# Autodesk Inventor assembly: RC_Car
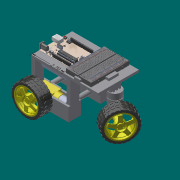
[picture p0: Inventor's stored thumbnail of the model, 180x180]
Saved by Autodesk Inventor 2019 (Build 230136000, 136)
## iProperties
Created: 2020-12-04
Part Number: RC_Car
Document SubType Name: Assembly
Designer: Jason
Mass: 430.82 g
Surface Area: 2607.9 cm^2
Volume: 430.82 cm^3
Density: 1 g/cm^3
Author: Jason
## Documents named in this file (11)
- D:\Inventor Files\RC_Car\RC_Car.iam
- D:\Inventor Files\RC_Car\Arduino Uno.ipt
- D:\Inventor Files\RC_Car\dc_motorl.ipt
- D:\Inventor Files\RC_Car\dc_wheel.ipt
- D:\Inventor Files\RC_Car\RC_Chassis.ipt
- D:\Inventor Files\RC_Car\breadboard_350_pos_asm.ipt
- D:\Inventor Files\RC_Car\BATTERY PACK BASE.ipt
- D:\Inventor Files\RC_Car\BATTERY PACK COVER.ipt
- D:\Inventor Files\RC_Car\Swing_Joint.ipt
- D:\Inventor Files\RC_Car\Swing_Joint_2.ipt
- D:\Inventor Files\RC_Car\Joint_Wheel_Connect.ipt
## Components (13 placed, 10 different names)
1. dc_motorl:1 — Mate:19, Flush:18, Mate:20, Insert:2
2. dc_motorl:2 — Flush:17, Mate:18, Mate:21, Insert:3
3. dc_wheel:2 — Insert:3
4. dc_wheel:3 — Insert:2
5. dc_wheel:1 — Mate:14, Mate:15, Mate:16
6. Arduino Uno:1 — Angle:6, Angle:7, Mate:24
7. BATTERY PACK COVER:1 — Mate:3, Mate:5, Mate:6, Mate:17, Flush:16
8. BATTERY PACK BASE:1 — Mate:3, Mate:5, Mate:6, Angle:6, Angle:7, Mate:23
9. breadboard_350_pos_asm:1 — Mate:9, Mate:10, Mate:22
10. RC_Chassis:1 — Mate:9, Mate:10, Flush:8, Flush:10, Mate:12, Flush:11, Mate:13, Mate:17, Flush:16, Flush:17, Mate:18, Mate:19, Flush:18, Mate:20, Mate:21, Mate:22, Mate:23, Mate:24
11. Swing_Joint:1 — Flush:8, Flush:10, Mate:12, Flush:11, Mate:13, Flush:12, Flush:13, Rotational:1
12. Swing_Joint_2:1 — Flush:12, Flush:13, Rotational:1, Flush:14, Flush:15
13. Joint_Wheel_Connect:1 — Flush:14, Flush:15, Mate:14, Mate:15, Mate:16
## Relationships (33: Mate 18, Flush 10, Angle 2, Insert 2, RevoluteJoint 1)
- Mate:3: BATTERY PACK COVER:1 ↔ BATTERY PACK BASE:1
- Mate:5: BATTERY PACK COVER:1 ↔ BATTERY PACK BASE:1
- Mate:6: BATTERY PACK COVER:1 ↔ BATTERY PACK BASE:1
- Angle:6 (0 deg): Arduino Uno:1 ↔ BATTERY PACK BASE:1
- Angle:7 (0 deg): Arduino Uno:1 ↔ BATTERY PACK BASE:1
- Mate:9: breadboard_350_pos_asm:1 ↔ RC_Chassis:1
- Mate:10: breadboard_350_pos_asm:1 ↔ RC_Chassis:1
- Flush:8: RC_Chassis:1 ↔ Swing_Joint:1
- Flush:10 (12.7 mm): RC_Chassis:1 ↔ Swing_Joint:1
- Mate:12: RC_Chassis:1 ↔ Swing_Joint:1
- Flush:11: RC_Chassis:1 ↔ Swing_Joint:1
- Mate:13: RC_Chassis:1 ↔ Swing_Joint:1
- Flush:12: Swing_Joint:1 ↔ Swing_Joint_2:1
- Flush:13: Swing_Joint:1 ↔ Swing_Joint_2:1
- Rotational:1 [RevoluteJoint]: Swing_Joint:1 ↔ Swing_Joint_2:1
- Flush:14: Swing_Joint_2:1 ↔ Joint_Wheel_Connect:1
- Flush:15: Swing_Joint_2:1 ↔ Joint_Wheel_Connect:1
- Mate:14: dc_wheel:1 ↔ Joint_Wheel_Connect:1
- Mate:15: dc_wheel:1 ↔ Joint_Wheel_Connect:1
- Mate:16: dc_wheel:1 ↔ Joint_Wheel_Connect:1
- Mate:17: BATTERY PACK COVER:1 ↔ RC_Chassis:1
- Flush:16 (12.7 mm): BATTERY PACK COVER:1 ↔ RC_Chassis:1
- Flush:17: dc_motorl:2 ↔ RC_Chassis:1
- Mate:18: dc_motorl:2 ↔ RC_Chassis:1
- Mate:19: dc_motorl:1 ↔ RC_Chassis:1
- Flush:18: dc_motorl:1 ↔ RC_Chassis:1
- Mate:20: dc_motorl:1 ↔ RC_Chassis:1
- Mate:21: dc_motorl:2 ↔ RC_Chassis:1
- Mate:22: breadboard_350_pos_asm:1 ↔ RC_Chassis:1
- Mate:23: BATTERY PACK BASE:1 ↔ RC_Chassis:1
- Mate:24: Arduino Uno:1 ↔ RC_Chassis:1
- Insert:2: dc_motorl:1 ↔ dc_wheel:3
- Insert:3: dc_motorl:2 ↔ dc_wheel:2
## Named parameters: sa_0 = -0, sa_1 = -2224.11, sa_2 = 4.44822e-13
note: some values were not read from the file. Shown as the stored number, unit unknown: "sa_0", "sa_1", "sa_2".
